# Autodesk Inventor assembly: ShoulderLeft
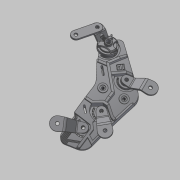
[picture p0: Inventor's stored thumbnail of the model, 180x180]
Saved by Autodesk Inventor 2015 SP1 (Build 190203100, 203)
## iProperties
Created: 2016-10-02
Part Number: ShoulderLeft
Document SubType Name: Assembly
Designer: Val
Author: Val
## Documents named in this file (7)
- C:\Users\Val\Desktop\ExoGit\elysium-max-exoskeleton\src\Assemblies\ShoulderLeft.iam
- C:\Users\Val\Desktop\ExoGit\elysium-max-exoskeleton\src\ShoulderLeft.ipt
- C:\Users\Val\Desktop\ExoGit\elysium-max-exoskeleton\src\ShoulderCogLarge.ipt
- C:\Users\Val\Desktop\ExoGit\elysium-max-exoskeleton\src\ShoulderCogSmall.ipt
- C:\Users\Val\Desktop\ExoGit\elysium-max-exoskeleton\src\BackConnector.ipt
- C:\Users\Val\Desktop\ExoGit\elysium-max-exoskeleton\src\BackSideConnector.ipt
- C:\Users\Val\Desktop\ExoGit\elysium-max-exoskeleton\src\Assemblies\ShoulderConnector.iam
## Components (10 placed, 6 different names)
1. ShoulderLeft:1 — Mate:1, Mate:2, Mate:3, Mate:4, Mate:5, Mate:6, Mate:7, Mate:8, Mate:9, Mate:10, Mate:13, Mate:15, Mate:17
2. ShoulderCogLarge:1 — Mate:1, Mate:2
3. ShoulderCogSmall:1 — Mate:7, Mate:8, Mate:14
4. ShoulderCogSmall:2 — Mate:5, Mate:6, Mate:16
5. ShoulderCogSmall:3 — Mate:3, Mate:4, Mate:18
6. BackConnector:1 — Mate:13, Mate:14
7. BackSideConnector:1 — Mate:11, Mate:12
8. BackConnector:2 — Mate:15, Mate:16
9. BackConnector:3 — Mate:17, Mate:18
10. ShoulderConnectorSplit:1 [sub-assembly] — Mate:9, Mate:10, Mate:11, Mate:12
## Relationships (18: Mate 18)
- Mate:1: ShoulderLeft:1 ↔ ShoulderCogLarge:1
- Mate:2: ShoulderLeft:1 ↔ ShoulderCogLarge:1
- Mate:3: ShoulderLeft:1 ↔ ShoulderCogSmall:3
- Mate:4: ShoulderLeft:1 ↔ ShoulderCogSmall:3
- Mate:5: ShoulderLeft:1 ↔ ShoulderCogSmall:2
- Mate:6: ShoulderLeft:1 ↔ ShoulderCogSmall:2
- Mate:7: ShoulderLeft:1 ↔ ShoulderCogSmall:1
- Mate:8: ShoulderLeft:1 ↔ ShoulderCogSmall:1
- Mate:9: ShoulderLeft:1 ↔ ShoulderConnectorSplit:1
- Mate:10: ShoulderLeft:1 ↔ ShoulderConnectorSplit:1
- Mate:11: BackSideConnector:1 ↔ ShoulderConnectorSplit:1
- Mate:12: BackSideConnector:1 ↔ ShoulderConnectorSplit:1
- Mate:13: ShoulderLeft:1 ↔ BackConnector:1
- Mate:14: ShoulderCogSmall:1 ↔ BackConnector:1
- Mate:15: ShoulderLeft:1 ↔ BackConnector:2
- Mate:16: ShoulderCogSmall:2 ↔ BackConnector:2
- Mate:17: ShoulderLeft:1 ↔ BackConnector:3
- Mate:18: ShoulderCogSmall:3 ↔ BackConnector:3
